# Autodesk Inventor assembly: PE4312-Enclosure
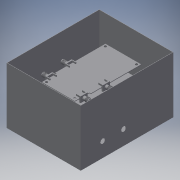
[picture p0: Inventor's stored thumbnail of the model, 180x180]
Saved by Autodesk Inventor 2018 (Build 220112000, 112)
## iProperties
Created: 2018-04-30
Part Number: PE4312-Enclosure
Document SubType Name: Assembly
Designer: bbramman
Author: bbramman
## Documents named in this file (4)
- C:\Users\bbramman\OneDrive\Documents\Trapped Ion Research (Grad)\Electronics\pll-evalboard-synthesizer\Box CAD\PE4312-Enclosure.iam
- C:\Users\bbramman\OneDrive\Documents\Trapped Ion Research (Grad)\Electronics\pll-evalboard-synthesizer\Box CAD\563-AU1028MG-PE4312.ipt
- C:\Users\bbramman\OneDrive\Documents\Trapped Ion Research (Grad)\Electronics\pll-evalboard-synthesizer\Box CAD\EV-PE4312-EK.iam
- C:\Users\bbramman\OneDrive\Documents\Trapped Ion Research (Grad)\Electronics\pll-evalboard-synthesizer\Box CAD\Power-Reg.iam
## Components (5 placed, 3 different names)
1. 563-AU1028MG-PE4312:1 — Insert:1, Insert:2, Mate:1, Mate:2
2. EV-PE4312-EK:1 [sub-assembly] — Insert:2
3. Power-Reg:1 [sub-assembly] — Insert:1
4. EV-PE4312-EK:2 [sub-assembly] — Mate:1
5. EV-PE4312-EK:3 [sub-assembly] — Mate:2
## Relationships (4: Insert 2, Mate 2)
- Insert:1 (-7.366 mm): 563-AU1028MG-PE4312:1 ↔ Power-Reg:1
- Insert:2 (19.05 mm): 563-AU1028MG-PE4312:1 ↔ EV-PE4312-EK:1
- Mate:1 (38.1 mm): 563-AU1028MG-PE4312:1 ↔ EV-PE4312-EK:2
- Mate:2 (57.15 mm): 563-AU1028MG-PE4312:1 ↔ EV-PE4312-EK:3
